# Autodesk Inventor assembly: NestArmFull-ver1-1111-2021
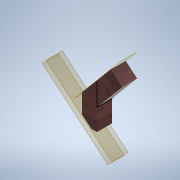
[picture p0: Inventor's stored thumbnail of the model, 180x180]
Saved by Autodesk Inventor 2021 (Build 250183000, 183)
## iProperties
Created: 2021-03-02
Part Number: NestArmFull-ver1-1111-2021
Document SubType Name: Assembly
Designer: CMurray
Author: CMurray
## Documents named in this file (3)
- F:\PHRC CADD 2021\2021 Game Design Challenge\Crow's Nest\Parts\NestArmFull-ver1-1111-2021.iam
- F:\PHRC CADD 2021\2021 Game Design Challenge\Crow's Nest\Parts\NestArmP1-ver1-1111-2021.ipt
- F:\PHRC CADD 2021\2021 Game Design Challenge\Crow's Nest\Parts\NestArmP2-ver1-1111-2021.ipt
## Components (2 placed, 2 different names)
1. NestArmP1-ver1-1111-2021:1 — Mate:1, Flush:1, Mate:3
2. NestArmP2-ver1-1111-2021:1 — Mate:1, Flush:1, Mate:2, Angle:1, Angle:2
## Relationships (7: Mate 3, Flush 2, Angle 2)
- Mate:1: NestArmP1-ver1-1111-2021:1 ↔ NestArmP2-ver1-1111-2021:1
- Flush:1: NestArmP1-ver1-1111-2021:1 ↔ NestArmP2-ver1-1111-2021:1
- Mate:2: NestArmP2-ver1-1111-2021:1
- Angle:1 (0 deg): NestArmP2-ver1-1111-2021:1
- Mate:3: NestArmP1-ver1-1111-2021:1
- Angle:2 (0 deg): NestArmP2-ver1-1111-2021:1
- Flush:2 (50.8 mm)
